# Autodesk Inventor assembly: Poliana-00.00-A01
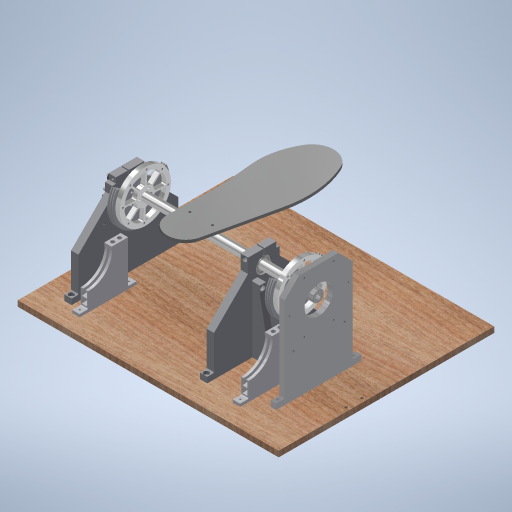
[picture p0: Inventor's stored thumbnail of the model, 512x512]
Saved by Autodesk Inventor 2023.2 (Build 272271000, 271)
## iProperties
Created: 2019-12-20
Part Number: Poliana-00.00-A01
Document SubType Name: Assembly
Designer: Barth
Author: Barth
## Documents named in this file (8)
- C:\Users\User\Desktop\CADs\Bancada\Poliana-00.00-A01.iam
- C:\Users\User\Desktop\CADs\Bancada\Poliana-01.05-A01.ipt
- C:\Users\User\Desktop\CADs\Bancada\Poliana-04.04-A01.ipt
- C:\Users\User\Desktop\CADs\Bancada\Poliana-04.06-A00.ipt
- C:\Users\User\Desktop\CADs\Bancada\Poliana-00.04-A01.iam
- C:\Users\User\Desktop\CADs\Bancada\Poliana-00.06-A02.iam
- C:\Users\User\Desktop\CADs\Bancada\ETMCAE-04.28-A00.iam
- C:\Users\User\Desktop\CADs\Bancada\suporte_motor.ipt
## Components (9 placed, 7 different names)
1. Poliana-01.05-A01:1 — Mate:10, Mate:12, Mate:13, Mate:14, Mate:21, Mate:31, Mate:33, Coincidente:36
2. Poliana-04.04-A01:1
3. Poliana-04.06-A00:1 — Mate:10
4. Poliana-00.04-A01:1 [sub-assembly] — Mate:12, Mate:13, Mate:14, Mate:17, Flush:1, Mate:18, Mate:19
5. Poliana-00.06-A02:1 [sub-assembly] — Mate:17, Flush:1, Mate:20, Flush:2, Mate:32, Coincidente:38
6. ETMCAE-04.28-A00:1 [sub-assembly] — Mate:18, Mate:19, Mate:20
7. Poliana-04.06-A00:2 — Mate:21, Flush:2
8. suporte_motor:1 — Coincidente:36, Coincidente:38
9. Poliana-00.04-A01:2 [sub-assembly] — Mate:31, Mate:32, Mate:33
## Relationships (16: Mate 14, Flush 2)
- Mate:10: Poliana-01.05-A01:1 ↔ Poliana-04.06-A00:1
- Mate:12: Poliana-01.05-A01:1 ↔ Poliana-00.04-A01:1
- Mate:13: Poliana-01.05-A01:1 ↔ Poliana-00.04-A01:1
- Mate:14: Poliana-01.05-A01:1 ↔ Poliana-00.04-A01:1
- Mate:17: Poliana-00.04-A01:1 ↔ Poliana-00.06-A02:1
- Flush:1: Poliana-00.04-A01:1 ↔ Poliana-00.06-A02:1
- Mate:18: Poliana-00.04-A01:1 ↔ ETMCAE-04.28-A00:1
- Mate:19: Poliana-00.04-A01:1 ↔ ETMCAE-04.28-A00:1
- Mate:20: Poliana-00.06-A02:1 ↔ ETMCAE-04.28-A00:1
- Mate:21: Poliana-01.05-A01:1 ↔ Poliana-04.06-A00:2
- Flush:2: Poliana-00.06-A02:1 ↔ Poliana-04.06-A00:2
- Mate:31: Poliana-01.05-A01:1 ↔ Poliana-00.04-A01:2
- Mate:32: Poliana-00.06-A02:1 ↔ Poliana-00.04-A01:2
- Mate:33: Poliana-01.05-A01:1 ↔ Poliana-00.04-A01:2
- Coincidente:36 [Mate]: Poliana-01.05-A01:1 ↔ suporte_motor:1
- Coincidente:38 [Mate] (25 mm): Poliana-00.06-A02:1 ↔ suporte_motor:1
